# Autodesk Inventor assembly: Belt Tensioner End_MIR2
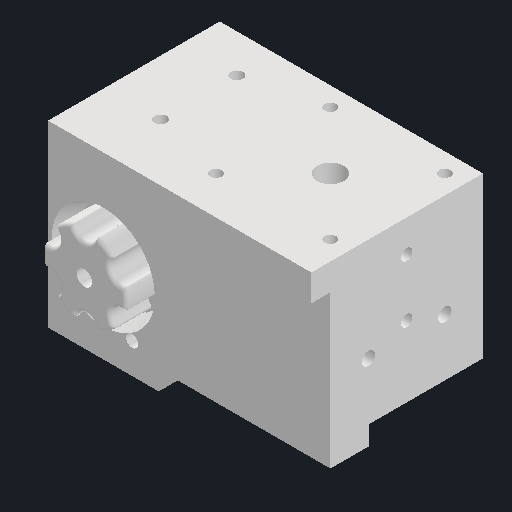
[picture p0: Inventor's stored thumbnail of the model, 512x512]
Saved by Autodesk Inventor 2026 (Build 300175000, 175)
## iProperties
Created: 2025-02-02
Part Number: Belt Tensioner End_MIR2
Document SubType Name: Assembly
Designer: jerem
Author: jerem
## Documents named in this file (7)
- C:\Users\jerem\Documents\GitHub\Perovskite-Automated-Synthesis-System\CAD\Gantry\X Axis\Belt Tensioner End_MIR.iam
- C:\Users\jerem\Documents\GitHub\Perovskite-Automated-Synthesis-System\CAD\Gantry\X Axis\Idlert Tensioner.ipt
- C:\Users\jerem\Documents\GitHub\Perovskite-Automated-Synthesis-System\CAD\Gantry\X Axis\Tensioner Holder.ipt
- C:\Users\jerem\Documents\GitHub\Perovskite-Automated-Synthesis-System\CAD\Gantry\X Axis\X Axis Rail End.ipt
- C:\Users\jerem\Documents\GitHub\Perovskite-Automated-Synthesis-System\CAD\Gantry\X Axis\Tensioner Top_MIR.ipt
- C:\Users\jerem\Documents\GitHub\Perovskite-Automated-Synthesis-System\CAD\Non 3D Printed Parts\Screws\M3x12.ipt
- C:\Users\jerem\Documents\GitHub\Perovskite-Automated-Synthesis-System\CAD\Gantry\X Axis\Tension Screw.ipt
## Components (6 placed, 6 different names)
1. Idlert Tensioner:1 — Angle:1, Mate:8, Angle:2, Mate:10, Mate:9
2. Tensioner Holder:1 — Angle:1, Mate:8, Angle:2, Mate:1, Flush:2, Flush:1, Mate:11
3. X Axis Rail End:1 — Mate:1, Flush:2, Flush:1, Mate:6, Mate:5, Mate:10
4. Tensioner Top_MIR:1 — Mate:6, Mate:5, Mate:10
5. M3x12:1 — Mate:10, Mate:9, Rotation/Translation:1, Mate:12
6. Tension Screw:1 — Rotation/Translation:1, Mate:12, Mate:11
## Relationships (14: Mate 9, Angle 2, Flush 2, RelateRotateTranslate 1)
- Angle:1 (180 deg): Idlert Tensioner:1 ↔ Tensioner Holder:1
- Mate:8: Idlert Tensioner:1 ↔ Tensioner Holder:1
- Angle:2 (0 deg): Idlert Tensioner:1 ↔ Tensioner Holder:1
- Mate:1: Tensioner Holder:1 ↔ X Axis Rail End:1
- Flush:2: Tensioner Holder:1 ↔ X Axis Rail End:1
- Flush:1: Tensioner Holder:1 ↔ X Axis Rail End:1
- Mate:6: X Axis Rail End:1 ↔ Tensioner Top_MIR:1
- Mate:5: X Axis Rail End:1 ↔ Tensioner Top_MIR:1
- Mate:10: Idlert Tensioner:1 ↔ M3x12:1
- Mate:9: Idlert Tensioner:1 ↔ M3x12:1
- Rotation/Translation:1 [RelateRotateTranslate] (10.996 mm): M3x12:1 ↔ Tension Screw:1
- Mate:12: M3x12:1 ↔ Tension Screw:1
- Mate:11: Tensioner Holder:1 ↔ Tension Screw:1
- Mate:10: X Axis Rail End:1 ↔ Tensioner Top_MIR:1
